# Autodesk Inventor assembly: PulleyAssembly
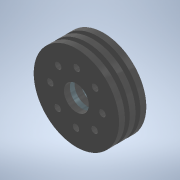
[picture p0: Inventor's stored thumbnail of the model, 180x180]
Saved by Autodesk Inventor 2020 (Build 240168000, 168)
## iProperties
Created: 2020-05-08
Part Number: PulleyAssembly
Document SubType Name: Assembly
Designer: Ajay Yadiki
Author: Ajay Yadiki
## Documents named in this file (3)
- C:\Users\Ajay Yadiki\Desktop\Project Gripper\PulleyAssembly.iam
- C:\Users\Ajay Yadiki\Desktop\Project Gripper\Pulley_base.ipt
- C:\Users\Ajay Yadiki\Desktop\Project Gripper\Pulley_middle.ipt
## Components (5 placed, 2 different names)
1. Pulley_base:1 — Mate:4, Mate:5, Mate:8, Mate:12
2. Pulley_base:2 — Mate:1, Mate:7, Mate:9
3. Pulley_base:3 — Mate:2, Mate:3, Mate:6, Mate:7, Mate:8, Mate:10, Mate:11
4. Pulley_middle:1 — Mate:1, Mate:3, Mate:6, Mate:9, Mate:10
5. Pulley_middle:2 — Mate:2, Mate:4, Mate:5, Mate:11, Mate:12
## Relationships (12: Mate 12)
- Mate:1: Pulley_base:2 ↔ Pulley_middle:1
- Mate:2: Pulley_base:3 ↔ Pulley_middle:2
- Mate:3: Pulley_base:3 ↔ Pulley_middle:1
- Mate:4: Pulley_base:1 ↔ Pulley_middle:2
- Mate:5: Pulley_base:1 ↔ Pulley_middle:2
- Mate:6: Pulley_base:3 ↔ Pulley_middle:1
- Mate:7: Pulley_base:2 ↔ Pulley_base:3
- Mate:8: Pulley_base:1 ↔ Pulley_base:3
- Mate:9: Pulley_base:2 ↔ Pulley_middle:1
- Mate:10: Pulley_base:3 ↔ Pulley_middle:1
- Mate:11: Pulley_base:3 ↔ Pulley_middle:2
- Mate:12: Pulley_base:1 ↔ Pulley_middle:2
